# Autodesk Inventor assembly: ciezarekztytkiem
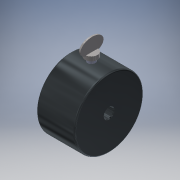
[picture p0: Inventor's stored thumbnail of the model, 180x180]
Saved by Autodesk Inventor 2019 (Build 230136000, 136)
## iProperties
Created: 2020-08-31
Part Number: ciezarekztytkiem
Document SubType Name: Assembly
Designer: estee
Author: estee
## Documents named in this file (3)
- C:\Users\estee\OneDrive\Pulpit\estere\1\MUM\wogoleNajnowszyGit\Mechanika\Moduł obrotu RET Estera\projejt\projejt\NoweZlozenie\ciezarekztytkiem.iam
- C:\Users\estee\OneDrive\Pulpit\estere\1\MUM\wogoleNajnowszyGit\Mechanika\Moduł obrotu RET Estera\projejt\projejt\NoweZlozenie\ciezarek.ipt
- C:\Users\estee\OneDrive\Pulpit\estere\1\MUM\wogoleNajnowszyGit\Mechanika\Moduł obrotu RET Estera\projejt\projejt\NoweZlozenie\Thumb Screw.ipt
## Components (2 placed, 2 different names)
1. ciezarek:1 — Tangent:1, Angle:1, Flush:1
2. Thumb Screw:1 — Tangent:1, Angle:1, Flush:1
## Relationships (3: Tangent 1, Angle 1, Flush 1)
- Tangent:1 (-20 mm): ciezarek:1 ↔ Thumb Screw:1
- Angle:1 (90 deg): ciezarek:1 ↔ Thumb Screw:1
- Flush:1 (25 mm): ciezarek:1 ↔ Thumb Screw:1
